# Autodesk Inventor assembly: Board
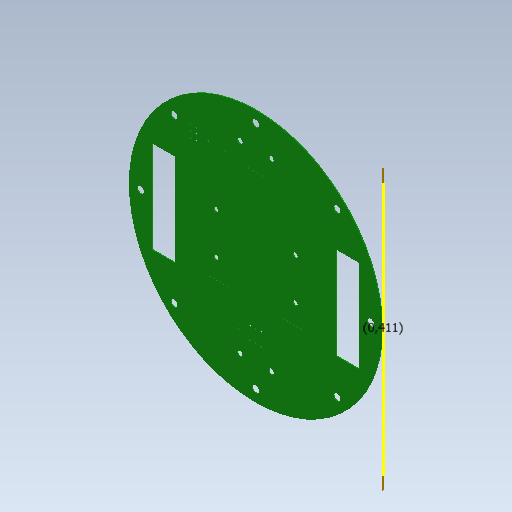
[picture p0: Inventor's stored thumbnail of the model, 512x512]
Saved by Autodesk Inventor 2020 (Build 240168000, 168)
## iProperties
Created: 2020-05-07
Part Number: Board
Document SubType Name: Assembly
Designer: jamnissa
Mass: 3.54107 g
Surface Area: 175.173 cm^2
Volume: 3.54107 cm^3
Density: 1 g/cm^3
Author: jamnissa
## Documents named in this file (2)
- C:\Users\jama1\Documents\GitHub\JRobots\pcbCase\Board\Board.iam
- C:\Users\jama1\Documents\GitHub\JRobots\pcbCase\Board\Open CASCADE STEP translator 6.8 1.1.1.ipt
## Components (1 placed, 1 different names)
1. Open CASCADE STEP translator 6.8 1.1.1_1 — Угол:1, Касательность:1
## Relationships (2: Angle 1, Tangent 1)
- Угол:1 [Angle] (0 deg): Open CASCADE STEP translator 6.8 1.1.1_1
- Касательность:1 [Tangent]: Open CASCADE STEP translator 6.8 1.1.1_1
